(part 1 of 2)
# Autodesk Inventor assembly: PumpConcept.Tube and Pipe Runs
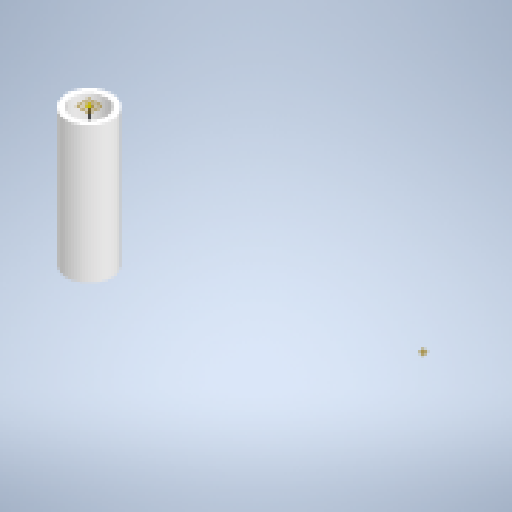
[picture p0: Inventor's stored thumbnail of the model, 512x512]
Saved by Autodesk Inventor 2025.2 (Build 292293000, 293)
## iProperties
Name: ISO 2531 - Flanged Ductile Iron Pipe and Fittings
ActiveState: False
PipeType: Rigid Pipe
RoutePreview: Solid
Material: UnInitValue
Standard: UnInitValue
FittingMaterial: UnInitValue
FittingStandard: UnInitValue
RouteDirection90: True
RouteDirection45: True
DiameterType: Nominal
Diameter: M40
Schedule: PN10
Ending: UnInitValue
IntermediateSegmentsMin: 1000 mm
IntermediateSegmentsMax: 9000 mm
IntermediateSegmentsInc: 10 mm
TerminationSegmentsMin: 1000 mm
TerminationSegmentsMax: 9000 mm
TerminationSegmentsInc: 10 mm
SolidRoutePreviewColor: 12632064
PipingComponentColor: As Material
PipeKey: v3#f52fbdcb-ece8-4303-8b76-5dbe8c7f2f9c#16
Elbow90Key: v3#451ae64e-c79d-4cba-b533-c09b8090ecb2#1
Elbow45Key: v3#81684a3f-f2a4-4fe6-95b1-f067ddead22f#1
_ComponentInfo: <CS><C N="Pipe" R="2.700000" IR="2.000000" PL="PL" PN="ISO 2531 Pipe with Integrally Cast Flanges DN40 PN 10"><CO N="1"><FE V="0"/><FD V="0"/><ET  V="Flanged"/><NS V="M40"/><MA V="0.000000"/><MI V="0.000000"/><WP X="0.000000" Y="-0.000000" Z="0.000000"/><WA X="1.000000" Y="0.000000"  Z="0.000000"/></CO><CO N="2"><FE V="0"/><FD V="1"/><ET V="Flanged"/><NS V="M40"/><MA V="0.000000"/><MI V="0.000000"/><WP X="-50.000000" Y="-0.000000"  Z="0.000000"/><WA X="1.000000" Y="0.000000" Z="0.000000"/></CO></C><C N="Elbow90" ER="14.000000" S1="14.000000" S2="14.000000" D1="0.000000"  D2="0.000000"><CO N="1"><FE V="0"/><FD V="0"/><ET V="Flanged"/><NS V="M40"/><MA V="0.000000"/><MI V="0.000000"/><WP X="14.000000" Y="0.000000"  Z="14.000000"/><WA X="1.000000" Y="0.000000" Z="0.000000"/></CO><CO N="2"><FE V="0"/><FD V="0"/><ET V="Flanged"/><NS V="M40"/><MA V="0.000000"/><MI  V="0.000000"/><WP X="0.000000" Y="0.000000" Z="0.000000"/><WA X="0.000000" Y="0.000000" Z="-1.000000"/></CO></C><C N="Elbow45" ER="33.798990"  S1="14.000000" S2="14.000000" D1="0.000000" D2="0.000000"><CO N="1"><FE V="0"/><FD V="0"/><ET V="Flanged"/><NS V="M40"/><MA V="0.000000"/><MI  V="0.000000"/><WP X="9.899495" Y="0.000000" Z="23.899495"/><WA X="0.707107" Y="0.000000" Z="0.707107"/></CO><CO N="2"><FE V="0"/><FD V="0"/><ET  V="Flanged"/><NS V="M40"/><MA V="0.000000"/><MI V="0.000000"/><WP X="-0.000000" Y="0.000000" Z="-0.000000"/><WA X="-0.000000" Y="0.000000"  Z="-1.000000"/></CO></C></CS>
BendRadius: UnInitValue
CategoryName: UnInitValue
DefaultBendRadius: 80 mm
EndFittingKey: UnInitValue
FlangeKey: UnInitValue
Gap: UnInitValue
GasketKey: UnInitValue
IsButtWelded: UnInitValue
IsFlanged: UnInitValue
MixedUnits: UnInitValue
RoundUpValue: UnInitValue
ShowGap: UnInitValue
StartFittingKey: UnInitValue
SuppressEndFitting: UnInitValue
SuppressStartFitting: UnInitValue
UseFlangsForCouplings: UnInitValue
UseSubASM: UnInitValue
Angle: UnInitValue
CustomFitElbow45Key: UnInitValue
CustomFitElbow90Key: UnInitValue
ElbowCustomKey: UnInitValue
IsSelfDraining: UnInitValue
PipingCustomFitElbowColor: UnInitValue
UseCustomFitElbows: UnInitValue
Name: Hydraulic Hose - Female Taper Thread
PipeType: Flexible Hose
RouteDirection90: UnInitValue
RouteDirection45: UnInitValue
Diameter: 1/2
Schedule: ID=0.5
OD: 2.235200000000000e+000
ID: 1.270000000000000e+000
IntermediateSegmentsMin: UnInitValue
IntermediateSegmentsMax: UnInitValue
IntermediateSegmentsInc: UnInitValue
TerminationSegmentsMin: UnInitValue
TerminationSegmentsMax: UnInitValue
TerminationSegmentsInc: UnInitValue
RoundUpValue: 0.125 in
PipeKey: v3#d489867e-ac9b-47ea-b952-0a1b885f66be#4
CouplingKey: UnInitValue
Elbow90Key: UnInitValue
Elbow45Key: UnInitValue
_ComponentInfo: <CS><C N="Pipe" R="1.117600" OR="1.117600" IR="0.635000" PL="PL" PartType="" SymKey="" PN="Parker Hydraulic Hose - No Skive 1/2"><CO N="1"><FE V="0"/><FD V="0"/><ET V="Hose - Permanent"/><NS V="1/2"/><MA V="2.540000"/><MI V="0.508000"/><WP X="12.700000" Y="0.000000" Z="0.000000"/><WA X="1.000000" Y="0.000000" Z="0.000000"/></CO><CO N="2"><FE V="0"/><FD V="1"/><ET V="Hose - Permanent"/><NS V="1/2"/><MA V="2.540000"/><MI V="0.508000"/><WP X="0.000000" Y="0.000000" Z="0.000000"/><WA X="1.000000" Y="0.000000" Z="0.000000"/></CO></C><C N="StartFitting" PartType="COUPLING" SymKey="COSC"><CO N="1"><FE V="1"/><FD V="1"/><ET V="Threaded"/><NS V="1/2"/><MA V="0.812800"/><MI V="0.162560"/><WP X="0.000000" Y="0.000000" Z="0.000000"/><WA X="1.000000" Y="-0.000000" Z="0.000000"/></CO><CO N="2"><FE V="1"/><FD V="0"/><ET V="Hose - Permanent"/><NS V="1/2"/><MA V="3.200400"/><MI V="3.200400"/><WP X="6.654800" Y="0.000000" Z="0.000000"/><WA X="1.000000" Y="-0.000000" Z="0.000000"/></CO></C><C N="EndFitting" PartType="COUPLING" SymKey="COSC"><CO N="1"><FE V="1"/><FD V="1"/><ET V="Threaded"/><NS V="1/2"/><MA V="0.812800"/><MI V="0.162560"/><WP X="0.000000" Y="0.000000" Z="0.000000"/><WA X="1.000000" Y="-0.000000" Z="0.000000"/></CO><CO N="2"><FE V="1"/><FD V="0"/><ET V="Hose - Permanent"/><NS V="1/2"/><MA V="3.200400"/><MI V="3.200400"/><WP X="6.654800" Y="0.000000" Z="0.000000"/><WA X="1.000000" Y="-0.000000" Z="0.000000"/></CO></C></CS>
BendRadius: 0.500 in
StartFittingKey: v3#cc3bd835-95a2-497d-9893-176cd9c426f6#7
EndFittingKey: v3#cc3bd835-95a2-497d-9893-176cd9c426f6#7
SuppressStartFitting: False
SuppressEndFitting: False
UseSubASM: True
DefaultBendRadius: UnInitValue
Name: JIS G 3458/JIS B 2316 -  Welded Steel Pipe and Fittings
Schedule: 80
IntermediateSegmentsMin: 60 mm
IntermediateSegmentsMax: 5000 mm
IntermediateSegmentsInc: 1 mm
TerminationSegmentsMin: 60 mm
TerminationSegmentsMax: 5000 mm
TerminationSegmentsInc: 1 mm
PipeKey: v3#da14b0ab-0b36-4851-8d66-8c9cd0bcbe86#23
CouplingKey: v3#12b64993-10e6-4915-8315-0c0cce209ad0#8
Elbow90Key: v3#1f65ece3-c41a-48d4-8661-909ed34ade86#8
Elbow45Key: v3#28e76e79-e22c-40ab-8be2-ff545b1407c5#8
_ComponentInfo: <CS><C N="Pipe" R="2.430000" IR="1.920000" PL="PL" PN="JIS G 3458 Pipe 40 A x Sch 80"><CO N="1"><FE V="0"/><FD V="1"/><ET V="Welded"/><NS  V="M40"/><MA V="0.000000"/><MI V="0.000000"/><WP X="0.000000" Y="0.000000" Z="0.000000"/><WA X="-1.000000" Y="0.000000" Z="0.000000"/></CO><CO  N="2"><FE V="0"/><FD V="0"/><ET V="Welded"/><NS V="M40"/><MA V="0.000000"/><MI V="0.000000"/><WP X="-25.000000" Y="0.000000" Z="0.000000"/><WA  X="-1.000000" Y="0.000000" Z="0.000000"/></CO></C><C N="Coupling" CW="3.810000"><CO N="1"><FE V="1"/><FD V="1"/><ET V="Welded"/><NS V="M40"/><MA  V="1.270000"/><MI V="0.254000"/><WP X="-0.000000" Y="0.000000" Z="0.000000"/><WA X="1.000000" Y="0.000000" Z="0.000000"/></CO><CO N="2"><FE  V="1"/><FD V="0"/><ET V="Welded"/><NS V="M40"/><MA V="1.270000"/><MI V="0.254000"/><WP X="3.810000" Y="0.000000" Z="0.000000"/><WA X="1.000000"  Y="0.000000" Z="0.000000"/></CO></C><C N="Elbow90" ER="3.180000" S1="4.450000" S2="4.450000" D1="1.270000" D2="1.270000"><CO N="1"><FE V="1"/><FD  V="1"/><ET V="Welded"/><NS V="M40"/><MA V="1.270000"/><MI V="0.254000"/><WP X="4.450000" Y="-0.000000" Z="4.450000"/><WA X="-1.000000" Y="0.000000"  Z="0.000000"/></CO><CO N="2"><FE V="1"/><FD V="1"/><ET V="Welded"/><NS V="M40"/><MA V="1.270000"/><MI V="0.254000"/><WP X="0.000000" Y="0.000000"  Z="0.000000"/><WA X="0.000000" Y="0.000000" Z="1.000000"/></CO></C><C N="Elbow45" ER="4.973280" S1="3.330000" S2="3.330000" D1="1.270000"  D2="1.270000"><CO N="1"><FE V="1"/><FD V="0"/><ET V="Welded"/><NS V="M40"/><MA V="1.270000"/><MI V="0.254000"/><WP X="2.354666" Y="0.000000"  Z="5.684666"/><WA X="0.707107" Y="0.000000" Z="0.707107"/></CO><CO N="2"><FE V="1"/><FD V="0"/><ET V="Welded"/><NS V="M40"/><MA V="1.270000"/><MI  V="0.254000"/><WP X="0.000000" Y="0.000000" Z="0.000000"/><WA X="0.000000" Y="0.000000" Z="-1.000000"/></CO></C></CS>
USE_R9_BOM: False
Name: Hydraulic Hose - SAE Flanged Connection
_ComponentInfo: <CS><C N="Pipe" R="1.117600" OR="1.117600" IR="0.635000" PL="PL" PartType="" SymKey="" PN="Parker Hydraulic Hose - No Skive 1/2"><CO N="1"><FE V="0"/><FD V="0"/><ET V="Hose - Permanent"/><NS V="1/2"/><MA V="2.540000"/><MI V="0.508000"/><WP X="12.700000" Y="0.000000" Z="0.000000"/><WA X="1.000000" Y="0.000000" Z="0.000000"/></CO><CO N="2"><FE V="0"/><FD V="1"/><ET V="Hose - Permanent"/><NS V="1/2"/><MA V="2.540000"/><MI V="0.508000"/><WP X="0.000000" Y="0.000000" Z="0.000000"/><WA X="1.000000" Y="0.000000" Z="0.000000"/></CO></C><C N="StartFitting" PartType="MISC-HYGENIC" SymKey="ADMF"><CO N="1"><FE V="0"/><FD V="1"/><ET V="Flanged"/><NS V="1/2"/><MA V="0.000000"/><MI V="0.000000"/><WP X="0.000000" Y="0.000000" Z="0.000000"/><WA X="1.000000" Y="0.000000" Z="0.000000"/></CO><CO N="2"><FE V="1"/><FD V="0"/><ET V="Hose - Permanent"/><NS V="1/2"/><MA V="3.200000"/><MI V="3.200000"/><WP X="8.800000" Y="0.000000" Z="0.000000"/><WA X="1.000000" Y="0.000000" Z="0.000000"/></CO></C><C N="EndFitting" PartType="MISC-HYGENIC" SymKey="ADMF"><CO N="1"><FE V="0"/><FD V="1"/><ET V="Flanged"/><NS V="1/2"/><MA V="0.000000"/><MI V="0.000000"/><WP X="0.000000" Y="0.000000" Z="0.000000"/><WA X="1.000000" Y="0.000000" Z="0.000000"/></CO><CO N="2"><FE V="1"/><FD V="0"/><ET V="Hose - Permanent"/><NS V="1/2"/><MA V="3.200000"/><MI V="3.200000"/><WP X="8.800000" Y="0.000000" Z="0.000000"/><WA X="1.000000" Y="0.000000" Z="0.000000"/></CO></C></CS>
StartFittingKey: v3#933069c9-73b6-4141-af99-628d4a97b2c2#1
EndFittingKey: v3#933069c9-73b6-4141-af99-628d4a97b2c2#1
DefaultBendRadius: 12 in
Diameter: 6
Elbow90Key: v3#97ecdcaf-8aa3-4fb0-8b6a-3da783de2ad5#108
Gap: 0.062 in
ID: UnInitValue
IntermediateSegmentsInc: 0.00001 in
IntermediateSegmentsMax: 200 in
IntermediateSegmentsMin: 3 in
IsButtWelded: True
IsFlanged: False
Name: ASTM A 53/A-ASME B16.9 - Steel Butt Welded Pipe
OD: UnInitValue
PipeKey: v3#4ce5e9fa-6da0-4801-ac02-ee7a0fb518d6#77
RouteDirection45: False
Schedule: 40
ShowGap: True
TerminationSegmentsInc: 0.00001 in
TerminationSegmentsMax: 200 in
TerminationSegmentsMin: 3 in
_ComponentInfo: <CS><C N="Elbow90" ER="15.240000" S1="15.240000" S2="15.240000" D1="0.000000" D2="0.000000" PartType="fitting" SymKey="ELBW"><CO N="1"><FE V="2"/><FD V="0"/><ET V="Butt Welded"/><NS V="6"/><MA V="0.000000"/><MI V="0.000000"/><WP X="15.240000" Y="0.000000" Z="15.240000"/><WA X="1.000000" Y="0.000000" Z="-0.000000"/></CO><CO N="2"><FE V="2"/><FD V="1"/><ET V="Butt Welded"/><NS V="6"/><MA V="0.000000"/><MI V="0.000000"/><WP X="0.000000" Y="0.000000" Z="0.000000"/><WA X="0.000000" Y="0.000000" Z="1.000000"/></CO></C><C N="Pipe" R="8.413750" OR="8.413750" IR="7.702550" PL="PL" PartType="pipe" SymKey="" PN="ASTM A 53/A 53M Pipe 6 - Schedule 40"><CO N="1"><FE V="2"/><FD V="0"/><ET V="Welded"/><NS V="6"/><MA V="0.000000"/><MI V="0.000000"/><WP X="25.400000" Y="0.000000" Z="0.000000"/><WA X="1.000000" Y="0.000000" Z="0.000000"/></CO><CO N="2"><FE V="2"/><FD V="1"/><ET V="Welded"/><NS V="6"/><MA V="0.000000"/><MI V="0.000000"/><WP X="0.000000" Y="0.000000" Z="0.000000"/><WA X="1.000000" Y="0.000000" Z="0.000000"/></CO></C></CS>
MixedUnits: False
Name: ASTM A53/A53M-ASME B16.11 - Welded Steel Pipe
Material: Steel
Standard: ASTM A 53/A 53M
FittingMaterial: Steel
FittingStandard: ASME B16.11
OD: Undefined
ID: Undefined
IntermediateSegmentsMin: 1 in
IntermediateSegmentsInc: 0.1 in
TerminationSegmentsMin: 1 in
TerminationSegmentsInc: 0.1 in
PipeKey: v3#4ce5e9fa-6da0-4801-ac02-ee7a0fb518d6#7
CouplingKey: v3#ed415c76-4cec-44a3-ba67-72e47bf70384#4
Elbow90Key: v3#82a08401-12d7-413b-b7f9-9cf3b607be7b#4
Elbow45Key: v3#2e5fd082-3851-4eb0-bde1-6c7078a7d72b#4
_ComponentInfo: <CS><C N="Pipe" R="1.066800" IR="0.789940" PL="PL" PN="ASTM A 53/A 53M Pipe 1/2 - Schedule 40"><CO N="1"><FE V="0"/><FD V="0"/><ET V="Welded"/><NS  V="1/2"/><MA V="0.000000"/><MI V="0.000000"/><WP X="25.400000" Y="0.000000" Z="0.000000"/><WA X="1.000000" Y="0.000000" Z="0.000000"/></CO><CO  N="2"><FE V="0"/><FD V="1"/><ET V="Welded"/><NS V="1/2"/><MA V="0.000000"/><MI V="0.000000"/><WP X="0.000000" Y="0.000000" Z="0.000000"/><WA  X="1.000000" Y="0.000000" Z="0.000000"/></CO></C><C N="Coupling" CW="2.895600"><CO N="1"><FE V="1"/><FD V="1"/><ET V="Welded"/><NS V="1/2"/><MA  V="0.965200"/><MI V="0.193040"/><WP X="-0.000000" Y="0.000000" Z="0.000000"/><WA X="1.000000" Y="0.000000" Z="0.000000"/></CO><CO N="2"><FE  V="1"/><FD V="0"/><ET V="Welded"/><NS V="1/2"/><MA V="0.965200"/><MI V="0.193040"/><WP X="2.895600" Y="0.000000" Z="0.000000"/><WA X="1.000000"  Y="0.000000" Z="0.000000"/></CO></C><C N="Elbow90" ER="1.574800" S1="2.540000" S2="2.540000" D1="0.965200" D2="0.965200"><CO N="1"><FE V="1"/><FD  V="1"/><ET V="Welded"/><NS V="1/2"/><MA V="0.965200"/><MI V="0.193040"/><WP X="2.540000" Y="0.000000" Z="2.540000"/><WA X="-1.000000" Y="0.000000"  Z="-0.000000"/></CO><CO N="2"><FE V="1"/><FD V="0"/><ET V="Welded"/><NS V="1/2"/><MA V="0.965200"/><MI V="0.193040"/><WP X="0.000000" Y="0.000000"  Z="0.000000"/><WA X="0.000000" Y="0.000000" Z="-1.000000"/></CO></C><C N="Elbow45" ER="2.698125" S1="2.082800" S2="2.082800" D1="0.965200"  D2="0.965200"><CO N="1"><FE V="1"/><FD V="0"/><ET V="Welded"/><NS V="1/2"/><MA V="0.965200"/><MI V="0.193040"/><WP X="1.472762" Y="0.000000"  Z="3.555562"/><WA X="0.707107" Y="0.000000" Z="0.707107"/></CO><CO N="2"><FE V="1"/><FD V="0"/><ET V="Welded"/><NS V="1/2"/><MA V="0.965200"/><MI  V="0.193040"/><WP X="0.000000" Y="0.000000" Z="0.000000"/><WA X="0.000000" Y="0.000000" Z="-1.000000"/></CO></C></CS>
DefaultBendRadius: 1 in
Name: ASTM D 1785-ASTM D 2466 - Jointed PVC Pipe and Fittings
ActiveState: True
Material: PVC-Piping
Standard: ASTM D 1785
FittingMaterial: PVC-Piping
FittingStandard: ASTM D 2466
IntermediateSegmentsMax: 100 in
TerminationSegmentsMax: 100 in
PipeKey: v3#4bf12049-4375-491b-8f13-d4ee0c517c57#1
CouplingKey: v3#29993622-4c6a-437e-8b8c-43a0846f8735#1
Elbow90Key: v3#25d2a8db-6517-4627-a5a4-9d27e4d26b9b#1
Elbow45Key: v3#d7b5d569-4a12-4d65-ba55-12203d6ac7ed#1
_ComponentInfo: <CS><C N="Pipe" R="1.066800" IR="0.789940" PL="PL" PN="ASTM D 1785 Pipe 1/2 - Schedule 40"><CO N="1"><FE V="0"/><FD V="0"/><ET V="Jointed"/><NS  V="1/2"/><MA V="2.540000"/><MI V="0.508000"/><WP X="127.000000" Y="0.000000" Z="0.000000"/><WA X="1.000000" Y="0.000000" Z="0.000000"/></CO><CO  N="2"><FE V="0"/><FD V="1"/><ET V="Jointed"/><NS V="1/2"/><MA V="2.540000"/><MI V="0.508000"/><WP X="0.000000" Y="0.000000" Z="0.000000"/><WA  X="1.000000" Y="0.000000" Z="0.000000"/></CO></C><C N="Coupling" CW="3.733165"><CO N="1"><FE V="1"/><FD V="0"/><ET V="Jointed"/><NS V="1/2"/><MA  V="1.747520"/><MI V="0.349504"/><WP X="3.733165" Y="0.000000" Z="0.000000"/><WA X="1.000000" Y="0.000000" Z="0.000000"/></CO><CO N="2"><FE V="1"/><FD  V="1"/><ET V="Jointed"/><NS V="1/2"/><MA V="1.747520"/><MI V="0.349504"/><WP X="0.000000" Y="0.000000" Z="0.000000"/><WA X="1.000000" Y="0.000000"  Z="0.000000"/></CO></C><C N="Elbow90" ER="1.270000" S1="3.017520" S2="3.017520" D1="1.747520" D2="1.747520"><CO N="1"><FE V="1"/><FD V="1"/><ET  V="Jointed"/><NS V="1/2"/><MA V="1.747520"/><MI V="0.349504"/><WP X="3.017520" Y="0.000000" Z="3.017520"/><WA X="-1.000000" Y="0.000000"  Z="-0.000000"/></CO><CO N="2"><FE V="1"/><FD V="1"/><ET V="Jointed"/><NS V="1/2"/><MA V="1.747520"/><MI V="0.349504"/><WP X="0.000000" Y="0.000000"  Z="0.000000"/><WA X="0.000000" Y="0.000000" Z="1.000000"/></CO></C><C N="Elbow45" ER="1.533026" S1="2.382520" S2="2.382520" D1="1.747520"  D2="1.747520"><CO N="1"><FE V="1"/><FD V="1"/><ET V="Jointed"/><NS V="1/2"/><MA V="1.747520"/><MI V="0.349504"/><WP X="1.684696" Y="0.000000"  Z="4.067216"/><WA X="-0.707107" Y="0.000000" Z="-0.707107"/></CO><CO N="2"><FE V="1"/><FD V="1"/><ET V="Jointed"/><NS V="1/2"/><MA V="1.747520"/><MI  V="0.349504"/><WP X="0.000000" Y="0.000000" Z="0.000000"/><WA X="0.000000" Y="0.000000" Z="1.000000"/></CO></C></CS>
Created: 2025-05-29
Part Number: PumpConcept.Tube and Pipe Runs
Document SubType Name: Tube & Pipe
Designer: Simon
Manufacturer: Standard
Standards Organization: Custom
Angle: 92.00 deg
DefaultBendRadius: 2 in
Diameter: 1
Elbow45Key: v3#bf26aa2a-f3dd-474c-8758-922a145c2b02#15
Elbow90Key: v3#3e93288f-9bb7-4e46-9d6b-544f8c20ca1c#3
ElbowCustomKey: v3#1f3bd44a-47ab-42f9-b3e0-74afa0c3f0ca#3
Gap: 0.094 in
IntermediateSegmentsMin: 2 in
IsSelfDraining: True
Name: ASME BPE - Butt Welded
PipeKey: v3#b10c956f-6fc6-429e-8056-0864a8581764#35
Schedule: ID=0.87
TerminationSegmentsMin: 2 in
_ComponentInfo: <CS><C N="Pipe" R="1.270000" OR="1.270000" IR="1.104900" PL="PL" PartType="pipe" SymKey="" PN="ASTM A 269 Tube with Welded ends 1 x 0.87"><CO N="1"><FE V="2"/><FD V="1"/><ET V="Welded"/><NS V="1"/><MA V="0.000000"/><MI V="0.000000"/><WP X="0.000000" Y="0.000000" Z="0.000000"/><WA X="1.000000" Y="0.000000" Z="0.000000"/></CO><CO N="2"><FE V="2"/><FD V="0"/><ET V="Welded"/><NS V="1"/><MA V="0.000000"/><MI V="0.000000"/><WP X="25.400000" Y="0.000000" Z="0.000000"/><WA X="1.000000" Y="0.000000" Z="0.000000"/></CO></C> <C N="Elbow90" ER="7.620000" S1="7.620000" S2="7.620000" D1="0.000000" D2="0.000000" PartType="fitting" SymKey="ELBW Elbow-Butt Weld(90 degree and 45 degree)"><CO N="1"><FE V="2"/><FD V="0"/><ET V="Butt Welded"/><NS V="1"/><MA V="0.000000"/><MI V="0.000000"/><WP X="0.000000" Y="0.000000" Z="0.000000"/><WA X="0.000000" Y="0.000000" Z="-1.000000"/></CO><CO N="2"><FE V="2"/><FD V="1"/><ET V="Butt Welded"/><NS V="1"/><MA V="0.000000"/><MI V="0.000000"/><WP X="0.000000" Y="7.620000" Z="7.620000"/><WA X="0.000000" Y="-1.000000" Z="0.000000"/></CO></C> <C N="Elbow45" ER="5.396250" S1="2.235200" S2="2.235200" D1="0.000000" D2="0.000000" PartType="fitting" SymKey="ELBW"><CO N="1"><FE V="2"/><FD V="0"/><ET V="Butt Welded"/><NS V="1"/><MA V="0.000000"/><MI V="0.000000"/><WP X="1.580525" Y="0.000000" Z="3.815725"/><WA X="0.707107" Y="0.000000" Z="0.707107"/></CO><CO N="2"><FE V="2"/><FD V="1"/><ET V="Butt Welded"/><NS V="1"/><MA V="0.000000"/><MI V="0.000000"/><WP X="0.000000" Y="0.000000" Z="0.000000"/><WA X="0.000000" Y="0.000000" Z="1.000000"/></CO></C> <C N="ElbowCustom" ER="7.746829" S1="7.485916" S2="7.481026" D1="0.004890" D2="0.000000" PartType="fitting" SymKey="ELBW Elbow-Butt Weld(90 degree and 45 degree)"><CO N="1"><FE V="2"/><FD V="1"/><ET V="Butt Welded"/><NS V="1"/><MA V="0.000000"/><MI V="0.000000"/><WP X="0.000000" Y="0.000000" Z="0.000000"/><WA X="0.000000" Y="-0.000000" Z="1.000000"/></CO><CO N="2"><FE V="2"/><FD V="0"/><ET V="Butt Welded"/><NS V="1"/><MA V="0.000000"/><MI V="0.000000"/><WP X="0.000000" Y="7.476469" Z="7.747000"/><WA X="0.000000" Y="0.999391" Z="0.034899"/></CO></C> </CS>
Elbow90Key: v3#6a678020-d9d9-4685-bba9-906b9a167083#10
FlangeKey: v3#c11442d2-c568-438f-a870-8ac9b5b636cb#10
GasketKey: v3#2a41914c-f5fb-4682-9c6a-1870d826d3d0#23
IsButtWelded: False
IsFlanged: True
Name: ASTM A 53/A-ASME B16.5 - Flanged Steel Threaded Pipe
PipeKey: v3#c5bd7d28-cdb3-4507-9f3d-c2787d93fe8a#40
_ComponentInfo: <CS><C N="Elbow90" ER="21.590000" S1="21.590000" S2="21.590000" D1="0.000000" D2="0.000000" PartType="fitting" SymKey="ELFL"><CO N="1"><FE V="2"/><FD V="1"/><ET V="Flanged"/><NS V="6"/><MA V="0.000000"/><MI V="0.000000"/><WP X="21.590000" Y="0.000000" Z="21.590000"/><WA X="-1.000000" Y="0.000000" Z="0.000000"/></CO><CO N="2"><FE V="2"/><FD V="0"/><ET V="Flanged"/><NS V="6"/><MA V="0.000000"/><MI V="0.000000"/><WP X="-0.000000" Y="0.000000" Z="-0.000000"/><WA X="-0.000000" Y="0.000000" Z="-1.000000"/></CO></C><C N="Gasket" CW="0.127000" PartType="fitting" SymKey=""><CO N="1"><FE V="2"/><FD V="1"/><ET V="Flanged"/><NS V="6"/><MA V="0.000000"/><MI V="0.000000"/><WP X="-0.000000" Y="0.127000" Z="0.000000"/><WA X="0.000000" Y="-1.000000" Z="0.000000"/></CO><CO N="2"><FE V="2"/><FD V="0"/><ET V="Flanged"/><NS V="6"/><MA V="0.000000"/><MI V="0.000000"/><WP X="-0.000000" Y="-0.000000" Z="0.000000"/><WA X="0.000000" Y="-1.000000" Z="0.000000"/></CO></C><C N="Pipe" R="8.413750" OR="8.413750" IR="7.702550" PL="PL" PartType="pipe" SymKey="" PN="ASTM A 53/A 53M Pipe with Threaded Ends 6 - Schedule 40"><CO N="1"><FE V="0"/><FD V="1"/><ET V="Threaded"/><NS V="6"/><MA V="3.206953"/><MI V="0.641391"/><WP X="7.683500" Y="0.000000" Z="0.000000"/><WA X="-1.000000" Y="0.000000" Z="-0.000000"/></CO><CO N="2"><FE V="0"/><FD V="0"/><ET V="Threaded"/><NS V="6"/><MA V="3.206953"/><MI V="0.641391"/><WP X="0.000000" Y="0.000000" Z="-0.000000"/><WA X="-1.000000" Y="0.000000" Z="-0.000000"/></CO></C><C N="Flange" CW="5.232400" PartType="fitting" SymKey="FLSC"><CO N="1"><FE V="2"/><FD V="1"/><ET V="Flanged"/><NS V="6"/><MA V="0.000000"/><MI V="0.000000"/><WP X="0.000000" Y="0.000000" Z="0.000000"/><WA X="1.000000" Y="0.000000" Z="0.000000"/></CO><CO N="2"><FE V="1"/><FD V="0"/><ET V="Threaded"/><NS V="6"/><MA V="5.232400"/><MI V="1.046480"/><WP X="5.232400" Y="0.000000" Z="0.000000"/><WA X="1.000000" Y="0.000000" Z="0.000000"/></CO></C> </CS>
IsSelfDraining: False
Name: ASME B36.10M-ASME B16.11 - Steel Threaded Pipe
Material: Wrought Steel
Standard: ASME B36.10M
Schedule: 30
OD: 2.1336
ID: 1.651
PipeKey: v3#4a736116-503a-44ad-a922-868ac6b46736#1
CouplingKey: v3#52ad3977-2b89-4007-a6a6-7626bac0ae85#4
Elbow90Key: v3#160eac10-3e6f-4b5c-839c-61eee0d373dc#4
Elbow45Key: v3#5c2ab816-abcb-49a6-a106-4733af000f51#4
_ComponentInfo: <CS><C N="Pipe" R="1.066800" IR="0.825500" PL="PL" PN="ASME B36.10M Pipe with Threaded Ends 1/2 - Schedule 30"><CO N="1"><FE V="0"/><FD V="1"/><ET  V="Threaded"/><NS V="1/2"/><MA V="1.355598"/><MI V="0.271120"/><WP X="25.400000" Y="0.000000" Z="-0.000000"/><WA X="-1.000000" Y="0.000000"  Z="0.000000"/></CO><CO N="2"><FE V="0"/><FD V="0"/><ET V="Threaded"/><NS V="1/2"/><MA V="1.355598"/><MI V="0.271120"/><WP X="0.000000" Y="0.000000"  Z="-0.000000"/><WA X="-1.000000" Y="0.000000" Z="0.000000"/></CO></C><C N="Coupling" CW="4.775200"><CO N="1"><FE V="1"/><FD V="0"/><ET  V="Threaded"/><NS V="1/2"/><MA V="1.355598"/><MI V="0.271120"/><WP X="4.775200" Y="0.000000" Z="0.000000"/><WA X="1.000000" Y="0.000000"  Z="0.000000"/></CO><CO N="2"><FE V="1"/><FD V="1"/><ET V="Threaded"/><NS V="1/2"/><MA V="1.355598"/><MI V="0.271120"/><WP X="0.000000" Y="0.000000"  Z="0.000000"/><WA X="1.000000" Y="0.000000" Z="0.000000"/></CO></C><C N="Elbow90" ER="1.971802" S1="3.327400" S2="3.327400" D1="1.355598"  D2="1.355598"><CO N="1"><FE V="1"/><FD V="1"/><ET V="Threaded"/><NS V="1/2"/><MA V="1.355598"/><MI V="0.271120"/><WP X="3.327400" Y="0.000000"  Z="3.327400"/><WA X="-1.000000" Y="0.000000" Z="0.000000"/></CO><CO N="2"><FE V="1"/><FD V="0"/><ET V="Threaded"/><NS V="1/2"/><MA V="1.355598"/><MI  V="0.271120"/><WP X="-0.000000" Y="0.000000" Z="0.000000"/><WA X="-0.000000" Y="0.000000" Z="-1.000000"/></CO></C><C N="Elbow45" ER="2.859399"  S1="2.540000" S2="2.540000" D1="1.355598" D2="1.355598"><CO N="1"><FE V="1"/><FD V="0"/><ET V="Threaded"/><NS V="1/2"/><MA V="1.355598"/><MI  V="0.271120"/><WP X="1.796051" Y="0.000000" Z="4.336051"/><WA X="0.707107" Y="0.000000" Z="0.707107"/></CO><CO N="2"><FE V="1"/><FD V="1"/><ET  V="Threaded"/><NS V="1/2"/><MA V="1.355598"/><MI V="0.271120"/><WP X="0.000000" Y="0.000000" Z="0.000000"/><WA X="0.000000" Y="0.000000"  Z="1.000000"/></CO></C></CS>
Name: DIN 2458/DIN 2605 - Welded Steel Pipe and Fittings
Schedule: ID=30.7
PipeKey: v3#dcef2839-8903-4c98-a96c-b861f5d9bb7f#98
Elbow90Key: v3#ace818b0-7b7c-4ad9-b19c-6da358a202c1#17
Elbow45Key: v3#97879d80-057e-491b-840b-74a9b3a7cf63#17
_ComponentInfo: <CS><C N="Pipe" R="2.415000" IR="1.535000" PL="PL" PN="DIN 2458 Pipe 48.3 x 8.8"><CO N="1"><FE V="2"/><FD V="0"/><ET V="Welded"/><NS V="M40"/><MA  V="0.000000"/><MI V="0.000000"/><WP X="25.000000" Y="0.000000" Z="0.000000"/><WA X="1.000000" Y="0.000000" Z="0.000000"/></CO><CO N="2"><FE  V="2"/><FD V="1"/><ET V="Welded"/><NS V="M40"/><MA V="0.000000"/><MI V="0.000000"/><WP X="0.000000" Y="0.000000" Z="0.000000"/><WA X="1.000000"  Y="0.000000" Z="0.000000"/></CO></C><C N="Elbow90" ER="3.800000" S1="3.800000" S2="3.800000" D1="0.000000" D2="0.000000"><CO N="1"><FE V="2"/><FD  V="1"/><ET V="Butt Welded"/><NS V="M40"/><MA V="0.000000"/><MI V="0.000000"/><WP X="0.000000" Y="0.000000" Z="0.000000"/><WA X="0.000000" Y="0.000000"  Z="1.000000"/></CO><CO N="2"><FE V="2"/><FD V="0"/><ET V="Butt Welded"/><NS V="M40"/><MA V="0.000000"/><MI V="0.000000"/><WP X="3.800000" Y="0.000000"  Z="3.800000"/><WA X="1.000000" Y="0.000000" Z="-0.000000"/></CO></C><C N="Elbow45" ER="3.862742" S1="1.600000" S2="1.600000" D1="0.000000"  D2="0.000000"><CO N="1"><FE V="2"/><FD V="1"/><ET V="Butt Welded"/><NS V="M40"/><MA V="0.000000"/><MI V="0.000000"/><WP X="0.000000" Y="0.000000"  Z="0.000000"/><WA X="0.000000" Y="0.000000" Z="1.000000"/></CO><CO N="2"><FE V="2"/><FD V="0"/><ET V="Butt Welded"/><NS V="M40"/><MA V="0.000000"/><MI  V="0.000000"/><WP X="1.131371" Y="0.000000" Z="2.731371"/><WA X="0.707107" Y="0.000000" Z="0.707107"/></CO></C></CS>
Name: Hydraulic Hose - Male Taper Thread
_ComponentInfo: <CS><C N="Pipe" R="1.117600" OR="1.117600" IR="0.635000" PL="PL" PartType="" SymKey="" PN="Parker Hydraulic Hose - No Skive 1/2"><CO N="1"><FE V="0"/><FD V="0"/><ET V="Hose - Permanent"/><NS V="1/2"/><MA V="2.540000"/><MI V="0.508000"/><WP X="12.700000" Y="0.000000" Z="0.000000"/><WA X="1.000000" Y="0.000000" Z="0.000000"/></CO><CO N="2"><FE V="0"/><FD V="1"/><ET V="Hose - Permanent"/><NS V="1/2"/><MA V="2.540000"/><MI V="0.508000"/><WP X="0.000000" Y="0.000000" Z="0.000000"/><WA X="1.000000" Y="0.000000" Z="0.000000"/></CO></C><C N="StartFitting" PartType="MISC-HYGENIC" SymKey="ADMF"><CO N="1"><FE V="0"/><FD V="1"/><ET V="Threaded"/><NS V="1/2"/><MA V="1.985010"/><MI V="0.397002"/><WP X="0.000000" Y="0.000000" Z="0.000000"/><WA X="1.000000" Y="0.000000" Z="0.000000"/></CO><CO N="2"><FE V="1"/><FD V="0"/><ET V="Hose - Permanent"/><NS V="1/2"/><MA V="3.200400"/><MI V="3.200400"/><WP X="7.213600" Y="0.000000" Z="0.000000"/><WA X="1.000000" Y="0.000000" Z="0.000000"/></CO></C><C N="EndFitting" PartType="MISC-HYGENIC" SymKey="ADMF"><CO N="1"><FE V="0"/><FD V="1"/><ET V="Threaded"/><NS V="1/2"/><MA V="1.985010"/><MI V="0.397002"/><WP X="0.000000" Y="0.000000" Z="0.000000"/><WA X="1.000000" Y="0.000000" Z="0.000000"/></CO><CO N="2"><FE V="1"/><FD V="0"/><ET V="Hose - Permanent"/><NS V="1/2"/><MA V="3.200400"/><MI V="3.200400"/><WP X="7.213600" Y="0.000000" Z="0.000000"/><WA X="1.000000" Y="0.000000" Z="0.000000"/></CO></C></CS>
StartFittingKey: v3#c8250148-a7b6-458b-b7bd-3b56763ca7cc#13
EndFittingKey: v3#c8250148-a7b6-458b-b7bd-3b56763ca7cc#13
Name: JIS G 3442/JIS B 2301 Threaded Steel Pipe and Iron Fittings
Schedule: ID=16.1
IntermediateSegmentsMin: 20 mm
TerminationSegmentsMin: 20 mm
PipeKey: v3#9964fba4-9d5a-4d75-85a8-e38022ccdce1#2
CouplingKey: v3#181262db-c004-4877-bc40-c64b931a44f6#3
Elbow90Key: v3#6c92b367-65e9-486b-b952-db434ae2548d#3
Elbow45Key: v3#960407aa-00b9-4d72-aae7-d50595845cfd#3
_ComponentInfo: <CS><C N="Pipe" R="1.085000" IR="0.805000" PL="PL" PN="JIS G 3442 Pipe with Threaded Ends 21.7 x 2.8"><CO N="1"><FE V="0"/><FD V="1"/><ET V="Threaded"/><NS V="1/2"/><MA V="1.316000"/><MI V="0.263200"/><WP X="25.000000" Y="0.000000" Z="-0.000000"/><WA X="-1.000000" Y="0.000000" Z="0.000000"/></CO><CO N="2"><FE V="0"/><FD V="0"/><ET V="Threaded"/><NS V="1/2"/><MA V="1.316000"/><MI V="0.263200"/><WP X="0.000000" Y="0.000000" Z="0.000000"/><WA X="-1.000000" Y="0.000000" Z="0.000000"/></CO></C><C N="Coupling" CW="3.500000"><CO N="1"><FE V="1"/><FD V="1"/><ET V="Threaded"/><NS V="1/2"/><MA V="1.100000"/><MI V="0.220000"/><WP X="0.000000" Y="-0.000000" Z="0.000000"/><WA X="1.000000" Y="0.000000" Z="0.000000"/></CO><CO N="2"><FE V="1"/><FD V="0"/><ET V="Threaded"/><NS V="1/2"/><MA V="1.100000"/><MI V="0.220000"/><WP X="3.500000" Y="0.000000" Z="0.000000"/><WA X="1.000000" Y="0.000000" Z="0.000000"/></CO></C><C N="Elbow90" ER="1.600000" S1="2.700000" S2="2.700000" D1="1.100000" D2="1.100000"><CO N="1"><FE V="1"/><FD V="0"/><ET V="Threaded"/><NS V="1/2"/><MA V="1.100000"/><MI V="0.220000"/><WP X="-0.000000" Y="0.000000" Z="-0.000000"/><WA X="-0.000000" Y="0.000000" Z="-1.000000"/></CO><CO N="2"><FE V="1"/><FD V="1"/><ET V="Threaded"/><NS V="1/2"/><MA V="1.100000"/><MI V="0.220000"/><WP X="2.700000" Y="0.000000" Z="2.700000"/><WA X="-1.000000" Y="0.000000" Z="0.000000"/></CO></C><C N="Elbow45" ER="2.414214" S1="2.100000" S2="2.100000" D1="1.100000" D2="1.100000"><CO N="1"><FE V="1"/><FD V="0"/><ET V="Threaded"/><NS V="1/2"/><MA V="1.100000"/><MI V="0.220000"/><WP X="0.000000" Y="0.000000" Z="0.000000"/><WA X="0.000000" Y="0.000000" Z="-1.000000"/></CO><CO N="2"><FE V="1"/><FD V="1"/><ET V="Threaded"/><NS V="1/2"/><MA V="1.100000"/><MI V="0.220000"/><WP X="1.484924" Y="0.000000" Z="3.584924"/><WA X="-0.707107" Y="0.000000" Z="-0.707107"/></CO></C></CS>
DefaultBendRadius: 25.4 mm
Name: ASTM B 88-ASME B16.22 - Soldered Copper Tubing
PipeType: Tubing
Material: Copper
Standard: ASTM B 88
FittingMaterial: *
FittingStandard: ASME B16.22
Schedule: L
IntermediateSegmentsMin: 0.000 in
IntermediateSegmentsMax: 100.000 in
IntermediateSegmentsInc: 0.100 in
TerminationSegmentsMin: 0.000 in
TerminationSegmentsMax: 100.000 in
TerminationSegmentsInc: 0.100 in
SolidRoutePreviewColor: 49344
PipeKey: v3#44b182c9-4bce-4825-bb4d-596143122252#7
CouplingKey: v3#0dc1ae02-7bbf-4ccf-8498-581434b0a765#3
_ComponentInfo: <CS><C N="Pipe" R="0.793750" IR="0.692150" PL="PL" PN="ASTM B 88 Tube 1/2 - Type L"><CO N="1"><FE V="0"/><FD V="0"/><ET V="Soldered"/><NS V="1/2"/><MA V="2.540000"/><MI V="0.508000"/><WP X="254.000000" Y="0.000000" Z="0.000000"/><WA X="1.000000" Y="0.000000" Z="0.000000"/></CO><CO N="2"><FE V="0"/><FD V="1"/><ET V="Soldered"/><NS V="1/2"/><MA V="2.540000"/><MI V="0.508000"/><WP X="0.000000" Y="0.000000" Z="0.000000"/><WA X="1.000000" Y="0.000000" Z="0.000000"/></CO></C><C N="Coupling" CW="2.540000"><CO N="1"><FE V="1"/><FD V="1"/><ET V="Soldered"/><NS V="1/2"/><MA V="1.270000"/><MI V="0.254000"/><WP X="2.540000" Y="0.000000" Z="-0.000000"/><WA X="-1.000000" Y="0.000000" Z="0.000000"/></CO><CO N="2"><FE V="1"/><FD V="0"/><ET V="Soldered"/><NS V="1/2"/><MA V="1.270000"/><MI V="0.254000"/><WP X="0.000000" Y="0.000000" Z="0.000000"/><WA X="-1.000000" Y="0.000000" Z="0.000000"/></CO></C></CS>
DefaultBendRadius: 2.000 in
CustomFitElbow90Key: v3#0eccf1d3-7418-433e-bb0f-cd3ee6f3b39a#119
Elbow90Key: v3#97ecdcaf-8aa3-4fb0-8b6a-3da783de2ad5#119
Name: ASTM A 53/A-ASME B16.9 - Steel Butt Welded Pipe (Custom Elbows)
UseCustomFitElbows: True
_ComponentInfo: <CS><C N="Pipe" R="8.413750" OR="8.413750" IR="7.702550" PL="PL" PartType="pipe" SymKey="" PN="ASTM A 53/A 53M Pipe 6 - Schedule 40"><CO N="1"><FE V="2"/><FD V="0"/><ET V="Welded"/><NS V="6"/><MA V="0.000000"/><MI V="0.000000"/><WP X="25.400000" Y="0.000000" Z="0.000000"/><WA X="1.000000" Y="0.000000" Z="0.000000"/></CO><CO N="2"><FE V="2"/><FD V="1"/><ET V="Welded"/><NS V="6"/><MA V="0.000000"/><MI V="0.000000"/><WP X="0.000000" Y="0.000000" Z="0.000000"/><WA X="1.000000" Y="0.000000" Z="0.000000"/></CO></C><C N="Elbow90" ER="15.240000" S1="15.240000" S2="15.240000" D1="0.000000" D2="0.000000" PartType="fitting" SymKey="ELBW"><CO N="1"><FE V="2"/><FD V="0"/><ET V="Butt Welded"/><NS V="6"/><MA V="0.000000"/><MI V="0.000000"/><WP X="15.240000" Y="0.000000" Z="15.240000"/><WA X="1.000000" Y="0.000000" Z="-0.000000"/></CO><CO N="2"><FE V="2"/><FD V="1"/><ET V="Butt Welded"/><NS V="6"/><MA V="0.000000"/><MI V="0.000000"/><WP X="0.000000" Y="0.000000" Z="0.000000"/><WA X="0.000000" Y="0.000000" Z="1.000000"/></CO></C> <C N="CustomFitElbow90" ER="15.240000" S1="15.240000" S2="15.240000" D1="0.000000" D2="0.000000" PartType="fitting" SymKey="ELBW"><CO N="1"><FE V="2"/><FD V="0"/><ET V="Butt Welded"/><NS V="6"/><MA V="0.000000"/><MI V="0.000000"/><WP X="15.240000" Y="0.000000" Z="15.240000"/><WA X="1.000000" Y="0.000000" Z="-0.000000"/></CO><CO N="2"><FE V="2"/><FD V="1"/><ET V="Butt Welded"/><NS V="6"/><MA V="0.000000"/><MI V="0.000000"/><WP X="0.000000" Y="0.000000" Z="0.000000"/><WA X="0.000000" Y="0.000000" Z="1.000000"/></CO></C> </CS>
PipingCustomFitElbowColor: As Material
FlangeKey: v3#24991861-26e3-4c21-a713-f46e314eddd5#10
Name: ASTM A 53/A 53M - Butt Welded/Flanged Steel Pipe
UseFlangsForCouplings: False
_ComponentInfo: <CS><C N="Pipe" R="8.413750" OR="8.413750" IR="7.702550" PL="PL" PartType="pipe" SymKey="" PN="ASTM A 53/A 53M Pipe 6 - Schedule 40"><CO N="1"><FE V="2"/><FD V="0"/><ET V="Welded"/><NS V="6"/><MA V="0.000000"/><MI V="0.000000"/><WP X="25.400000" Y="0.000000" Z="0.000000"/><WA X="1.000000" Y="0.000000" Z="0.000000"/></CO><CO N="2"><FE V="2"/><FD V="1"/><ET V="Welded"/><NS V="6"/><MA V="0.000000"/><MI V="0.000000"/><WP X="0.000000" Y="0.000000" Z="0.000000"/><WA X="1.000000" Y="0.000000" Z="0.000000"/></CO></C> <C N="Elbow90" ER="21.590000" S1="21.590000" S2="21.590000" D1="0.000000" D2="0.000000" PartType="fitting" SymKey="ELFL"><CO N="1"><FE V="2"/><FD V="1"/><ET V="Flanged"/><NS V="6"/><MA V="0.000000"/><MI V="0.000000"/><WP X="21.590000" Y="0.000000" Z="21.590000"/><WA X="-1.000000" Y="0.000000" Z="0.000000"/></CO><CO N="2"><FE V="2"/><FD V="0"/><ET V="Flanged"/><NS V="6"/><MA V="0.000000"/><MI V="0.000000"/><WP X="-0.000000" Y="0.000000" Z="-0.000000"/><WA X="-0.000000" Y="0.000000" Z="-1.000000"/></CO></C> <C N="Gasket" CW="0.127000" PartType="fitting" SymKey=""><CO N="1"><FE V="2"/><FD V="1"/><ET V="Flanged"/><NS V="6"/><MA V="0.000000"/><MI V="0.000000"/><WP X="-0.000000" Y="0.127000" Z="0.000000"/><WA X="0.000000" Y="-1.000000" Z="0.000000"/></CO><CO N="2"><FE V="2"/><FD V="0"/><ET V="Flanged"/><NS V="6"/><MA V="0.000000"/><MI V="0.000000"/><WP X="-0.000000" Y="-0.000000" Z="0.000000"/><WA X="0.000000" Y="-1.000000" Z="0.000000"/></CO></C> <C N="Flange" CW="9.855200" PartType="fitting" SymKey="FLWN"><CO N="1"><FE V="2"/><FD V="1"/><ET V="Flanged"/><NS V="6"/><MA V="0.000000"/><MI V="0.000000"/><WP X="0.000000" Y="-0.000000" Z="0.000000"/><WA X="1.000000" Y="0.000000" Z="0.000000"/></CO><CO N="2"><FE V="2"/><FD V="0"/><ET V="Butt Welded"/><NS V="6"/><MA V="0.000000"/><MI V="0.000000"/><WP X="9.855200" Y="0.000000" Z="0.000000"/><WA X="1.000000" Y="0.000000" Z="0.000000"/></CO></C> </CS>
Name: ISO 7598/ISO 49 - Threaded Steel Pipe with Iron Fittings
IntermediateSegmentsMin: 50.8 mm
IntermediateSegmentsMax: 5080 mm
IntermediateSegmentsInc: 2.54 mm
TerminationSegmentsMin: 50.8 mm
TerminationSegmentsMax: 5080 mm
TerminationSegmentsInc: 2.54 mm
PipeKey: v3#1052637f-74b5-47f4-adeb-d4e8d3fa53b8#1
CouplingKey: v3#7e56b2cb-a132-4546-b8a7-a14538454b94#3
Elbow90Key: v3#b72bb08b-ad33-47cc-a03d-7f3d76c6616b#3
Elbow45Key: v3#a96c5204-26e4-4bb2-b8f1-f0623fbc94bb#2
_ComponentInfo: <CS><C N="Pipe" R="1.065000" IR="0.805000" PL="PL" PN="ISO 7598 Tube with Threaded Ends DN15"><CO N="1"><FE V="0"/><FD V="1"/><ET V="Threaded"/><NS V="1/2"/><MA V="1.316000"/><MI V="0.263200"/><WP X="25.000000" Y="0.000000" Z="-0.000000"/><WA X="-1.000000" Y="0.000000" Z="0.000000"/></CO><CO N="2"><FE V="0"/><FD V="0"/><ET V="Threaded"/><NS V="1/2"/><MA V="1.316000"/><MI V="0.263200"/><WP X="0.000000" Y="0.000000" Z="0.000000"/><WA X="-1.000000" Y="0.000000" Z="0.000000"/></CO></C><C N="Coupling" CW="3.600000"><CO N="1"><FE V="1"/><FD V="0"/><ET V="Threaded"/><NS V="1/2"/><MA V="1.300000"/><MI V="0.260000"/><WP X="3.600000" Y="0.000000" Z="0.000000"/><WA X="1.000000" Y="0.000000" Z="0.000000"/></CO><CO N="2"><FE V="1"/><FD V="1"/><ET V="Threaded"/><NS V="1/2"/><MA V="1.300000"/><MI V="0.260000"/><WP X="-0.000000" Y="0.000000" Z="0.000000"/><WA X="1.000000" Y="-0.000000" Z="0.000000"/></CO></C><C N="Elbow90" ER="4.200000" S1="5.500000" S2="5.500000" D1="1.300000" D2="1.300000"><CO N="1"><FE V="1"/><FD V="1"/><ET V="Threaded"/><NS V="1/2"/><MA V="1.300000"/><MI V="0.260000"/><WP X="5.500000" Y="0.000000" Z="5.500000"/><WA X="-1.000000" Y="0.000000" Z="0.000000"/></CO><CO N="2"><FE V="1"/><FD V="0"/><ET V="Threaded"/><NS V="1/2"/><MA V="1.300000"/><MI V="0.260000"/><WP X="-0.000000" Y="0.000000" Z="-0.000000"/><WA X="-0.000000" Y="0.000000" Z="-1.000000"/></CO></C><C N="Elbow45" ER="5.552691" S1="3.600000" S2="3.600000" D1="1.300000" D2="1.300000"><CO N="1"><FE V="1"/><FD V="1"/><ET V="Threaded"/><NS V="1/2"/><MA V="1.300000"/><MI V="0.260000"/><WP X="2.545584" Y="0.000000" Z="6.145584"/><WA X="-0.707107" Y="0.000000" Z="-0.707107"/></CO><CO N="2"><FE V="1"/><FD V="0"/><ET V="Threaded"/><NS V="1/2"/><MA V="1.300000"/><MI V="0.260000"/><WP X="-0.000000" Y="0.000000" Z="-0.000000"/><WA X="-0.000000" Y="0.000000" Z="-1.000000"/></CO></C></CS>
Name: ANSI/ASME B36.19M-ASME B16.3 - Threaded Pipe with Iron Fittings
Material: Stainless Steel
Standard: ANSI/ASME B36.19M
FittingMaterial: Malleable Iron
FittingStandard: ASME B16.3
Schedule: 40S
PipeKey: v3#323c0148-c750-449d-a0c6-11721f2a5046#1
CouplingKey: v3#771d4942-b9e7-43bc-9d41-ab12a9580492#3
Elbow90Key: v3#bc6b44ab-9235-4590-b699-74498030a1ff#3
Elbow45Key: v3#626cc28c-1a24-4045-be0d-40d896dc828d#3
_ComponentInfo: <CS><C N="Pipe" R="1.066800" IR="0.789940" PL="PL" PN="ANSI/ASME B36.19M Pipe with Threaded Ends 1/2 - Schedule 40S"><CO N="1"><FE V="0"/><FD  V="1"/><ET V="Threaded"/><NS V="1/2"/><MA V="1.355598"/><MI V="0.271120"/><WP X="25.400000" Y="0.000000" Z="-0.000000"/><WA X="-1.000000"  Y="0.000000" Z="0.000000"/></CO><CO N="2"><FE V="0"/><FD V="0"/><ET V="Threaded"/><NS V="1/2"/><MA V="1.355598"/><MI V="0.271120"/><WP X="0.000000"  Y="0.000000" Z="-0.000000"/><WA X="-1.000000" Y="0.000000" Z="0.000000"/></CO></C><C N="Coupling" CW="3.403600"><CO N="1"><FE V="1"/><FD V="0"/><ET  V="Threaded"/><NS V="1/2"/><MA V="1.092200"/><MI V="0.218440"/><WP X="3.403600" Y="-0.000000" Z="0.000000"/><WA X="1.000000" Y="-0.000000"  Z="0.000000"/></CO><CO N="2"><FE V="1"/><FD V="1"/><ET V="Threaded"/><NS V="1/2"/><MA V="1.092200"/><MI V="0.218440"/><WP X="0.000000" Y="-0.000000"  Z="0.000000"/><WA X="1.000000" Y="-0.000000" Z="0.000000"/></CO></C><C N="Elbow90" ER="1.752600" S1="2.844800" S2="2.844800" D1="1.092200"  D2="1.092200"><CO N="1"><FE V="1"/><FD V="1"/><ET V="Threaded"/><NS V="1/2"/><MA V="1.092200"/><MI V="0.218440"/><WP X="2.844800" Y="0.000000"  Z="2.844800"/><WA X="-1.000000" Y="0.000000" Z="0.000000"/></CO><CO N="2"><FE V="1"/><FD V="0"/><ET V="Threaded"/><NS V="1/2"/><MA V="1.092200"/><MI  V="0.218440"/><WP X="0.000000" Y="0.000000" Z="-0.000000"/><WA X="-0.000000" Y="0.000000" Z="-1.000000"/></CO></C><C N="Elbow45" ER="2.759446"  S1="2.235200" S2="2.235200" D1="1.092200" D2="1.092200"><CO N="1"><FE V="1"/><FD V="1"/><ET V="Threaded"/><NS V="1/2"/><MA V="1.092200"/><MI  V="0.218440"/><WP X="1.580525" Y="0.000000" Z="3.815725"/><WA X="-0.707107" Y="0.000000" Z="-0.707107"/></CO><CO N="2"><FE V="1"/><FD V="0"/><ET  V="Threaded"/><NS V="1/2"/><MA V="1.092200"/><MI V="0.218440"/><WP X="0.000000" Y="0.000000" Z="-0.000000"/><WA X="-0.000000" Y="0.000000"  Z="-1.000000"/></CO></C></CS>
Name: DIN 2458/DIN EN 10242 - Threaded Steel Pipe and Iron Fittings
Schedule: ID=12.3
PipeKey: v3#d689fd5f-ac5a-46d7-a883-3089b2f6e0a4#28
CouplingKey: v3#d2599e7a-1865-48da-a234-5418a1cd5dfe#3
Elbow90Key: v3#9fba244e-81ed-4fc6-a9ac-7eb372fa3ffe#3
Elbow45Key: v3#6ce5b1be-37aa-4928-b23a-0df64e6ddf38#2
_ComponentInfo: <CS><C N="Pipe" R="1.065000" IR="0.615000" PL="PL" PN="DIN 2458 Pipe with Threaded Ends 21.3 x 4.5"><CO N="1"><FE V="0"/><FD V="1"/><ET V="Threaded"/><NS V="1/2"/><MA V="1.372000"/><MI V="0.274400"/><WP X="25.000000" Y="0.000000" Z="-0.000000"/><WA X="-1.000000" Y="0.000000" Z="0.000000"/></CO><CO N="2"><FE V="0"/><FD V="0"/><ET V="Threaded"/><NS V="1/2"/><MA V="1.372000"/><MI V="0.274400"/><WP X="-0.000000" Y="0.000000" Z="-0.000000"/><WA X="-1.000000" Y="0.000000" Z="0.000000"/></CO></C><C N="Coupling" CW="3.600000"><CO N="1"><FE V="1"/><FD V="1"/><ET V="Threaded"/><NS V="1/2"/><MA V="1.300000"/><MI V="0.260000"/><WP X="0.000000" Y="0.000000" Z="0.000000"/><WA X="1.000000" Y="0.000000" Z="0.000000"/></CO><CO N="2"><FE V="1"/><FD V="0"/><ET V="Threaded"/><NS V="1/2"/><MA V="1.300000"/><MI V="0.260000"/><WP X="3.600000" Y="0.000000" Z="0.000000"/><WA X="1.000000" Y="0.000000" Z="0.000000"/></CO></C><C N="Elbow90" ER="4.200000" S1="5.500000" S2="5.500000" D1="1.300000" D2="1.300000"><CO N="1"><FE V="1"/><FD V="0"/><ET V="Threaded"/><NS V="1/2"/><MA V="1.300000"/><MI V="0.260000"/><WP X="-0.000000" Y="0.000000" Z="-0.000000"/><WA X="-0.000000" Y="0.000000" Z="-1.000000"/></CO><CO N="2"><FE V="1"/><FD V="1"/><ET V="Threaded"/><NS V="1/2"/><MA V="1.300000"/><MI V="0.260000"/><WP X="5.500000" Y="0.000000" Z="5.500000"/><WA X="-1.000000" Y="0.000000" Z="0.000000"/></CO></C><C N="Elbow45" ER="5.552691" S1="3.600000" S2="3.600000" D1="1.300000" D2="1.300000"><CO N="1"><FE V="1"/><FD V="1"/><ET V="Threaded"/><NS V="1/2"/><MA V="1.300000"/><MI V="0.260000"/><WP X="2.545584" Y="0.000000" Z="6.145584"/><WA X="-0.707107" Y="0.000000" Z="-0.707107"/></CO><CO N="2"><FE V="1"/><FD V="0"/><ET V="Threaded"/><NS V="1/2"/><MA V="1.300000"/><MI V="0.260000"/><WP X="-0.000000" Y="0.000000" Z="-0.000000"/><WA X="-0.000000" Y="0.000000" Z="-1.000000"/></CO></C></CS>
Name: Hydraulic Hose - Female Thread - Swivel
_ComponentInfo: <CS><C N="Pipe" R="1.117600" OR="1.117600" IR="0.635000" PL="PL" PartType="" SymKey="" PN="Parker Hydraulic Hose - No Skive 1/2"><CO N="1"><FE V="0"/><FD V="0"/><ET V="Hose - Permanent"/><NS V="1/2"/><MA V="2.540000"/><MI V="0.508000"/><WP X="12.700000" Y="0.000000" Z="0.000000"/><WA X="1.000000" Y="0.000000" Z="0.000000"/></CO><CO N="2"><FE V="0"/><FD V="1"/><ET V="Hose - Permanent"/><NS V="1/2"/><MA V="2.540000"/><MI V="0.508000"/><WP X="0.000000" Y="0.000000" Z="0.000000"/><WA X="1.000000" Y="0.000000" Z="0.000000"/></CO></C><C N="StartFitting" PartType="COUPLING" SymKey="COSC"><CO N="1"><FE V="1"/><FD V="1"/><ET V="Threaded"/><NS V="3/4-16 UNF"/><MA V="0.970000"/><MI V="0.194000"/><WP X="-0.000000" Y="0.000000" Z="0.000000"/><WA X="1.000000" Y="0.000000" Z="0.000000"/></CO><CO N="2"><FE V="1"/><FD V="0"/><ET V="Hose - Permanent"/><NS V="1/2"/><MA V="3.470000"/><MI V="3.470000"/><WP X="6.650000" Y="0.000000" Z="0.000000"/><WA X="1.000000" Y="0.000000" Z="0.000000"/></CO></C><C N="EndFitting" PartType="COUPLING" SymKey="COSC"><CO N="1"><FE V="1"/><FD V="1"/><ET V="Threaded"/><NS V="3/4-16 UNF"/><MA V="0.970000"/><MI V="0.194000"/><WP X="-0.000000" Y="0.000000" Z="0.000000"/><WA X="1.000000" Y="0.000000" Z="0.000000"/></CO><CO N="2"><FE V="1"/><FD V="0"/><ET V="Hose - Permanent"/><NS V="1/2"/><MA V="3.470000"/><MI V="3.470000"/><WP X="6.650000" Y="0.000000" Z="0.000000"/><WA X="1.000000" Y="0.000000" Z="0.000000"/></CO></C></CS>
StartFittingKey: v3#c5e461f5-5e73-4f2e-8c1e-4358d4d6f46c#4
EndFittingKey: v3#c5e461f5-5e73-4f2e-8c1e-4358d4d6f46c#4
Name: JIS K 6741/JIS K 6739 - Jointed PVC-U Pipe and Fittings
Schedule: VP
IntermediateSegmentsMax: 2500 mm
TerminationSegmentsMax: 2500 mm
PipeKey: v3#45338dd0-af69-48c0-a2ed-8ade33a08701#5
CouplingKey: v3#eaa8de87-dc67-4eca-ba7e-4267a30f8f7f#2
Elbow90Key: v3#c4513a61-3106-4a78-baf9-a1badd100245#2
Elbow45Key: v3#2769403e-a4fd-4a4c-8e4c-659ea845bd78#2
_ComponentInfo: <CS><C N="Pipe" R="2.400000" IR="2.040000" PL="PL" PN="JIS K 6741 Pipe VP 40"><CO N="1"><FE V="0"/><FD V="1"/><ET V="Jointed"/><NS V="M40"/><MA  V="4.000000"/><MI V="0.800000"/><WP X="0.000000" Y="0.000000" Z="0.000000"/><WA X="-1.000000" Y="0.000000" Z="0.000000"/></CO><CO N="2"><FE  V="0"/><FD V="0"/><ET V="Jointed"/><NS V="M40"/><MA V="4.000000"/><MI V="0.800000"/><WP X="-25.000000" Y="0.000000" Z="0.000000"/><WA X="-1.000000"  Y="0.000000" Z="0.000000"/></CO></C><C N="Coupling" CW="4.700000"><CO N="1"><FE V="1"/><FD V="1"/><ET V="Jointed"/><NS V="M40"/><MA V="2.200000"/><MI  V="0.440000"/><WP X="0.000000" Y="0.000000" Z="0.000000"/><WA X="1.000000" Y="0.000000" Z="0.000000"/></CO><CO N="2"><FE V="1"/><FD V="0"/><ET  V="Jointed"/><NS V="M40"/><MA V="2.200000"/><MI V="0.440000"/><WP X="4.700000" Y="0.000000" Z="0.000000"/><WA X="1.000000" Y="0.000000"  Z="0.000000"/></CO></C><C N="Elbow90" ER="2.700000" S1="4.900000" S2="4.900000" D1="2.200000" D2="2.200000"><CO N="1"><FE V="1"/><FD V="1"/><ET  V="Jointed"/><NS V="M40"/><MA V="2.200000"/><MI V="0.440000"/><WP X="4.900000" Y="0.000000" Z="4.900000"/><WA X="-1.000000" Y="0.000000"  Z="0.000000"/></CO><CO N="2"><FE V="1"/><FD V="0"/><ET V="Jointed"/><NS V="M40"/><MA V="2.200000"/><MI V="0.440000"/><WP X="0.000000" Y="0.000000"  Z="0.000000"/><WA X="0.000000" Y="0.000000" Z="-1.000000"/></CO></C><C N="Elbow45" ER="3.379899" S1="3.600000" S2="3.600000" D1="2.200000"  D2="2.200000"><CO N="1"><FE V="1"/><FD V="1"/><ET V="Jointed"/><NS V="M40"/><MA V="2.200000"/><MI V="0.440000"/><WP X="2.545584" Y="0.000000"  Z="6.145584"/><WA X="-0.707107" Y="0.000000" Z="-0.707107"/></CO><CO N="2"><FE V="1"/><FD V="0"/><ET V="Jointed"/><NS V="M40"/><MA V="2.200000"/><MI  V="0.440000"/><WP X="0.000000" Y="0.000000" Z="0.000000"/><WA X="0.000000" Y="0.000000" Z="-1.000000"/></CO></C></CS>
Name: Hydraulic Hose - Male Straight Thread
_ComponentInfo: <CS><C N="Pipe" R="1.117600" OR="1.117600" IR="0.635000" PL="PL" PartType="" SymKey="" PN="Parker Hydraulic Hose - No Skive 1/2"><CO N="1"><FE V="0"/><FD V="0"/><ET V="Hose - Permanent"/><NS V="1/2"/><MA V="2.540000"/><MI V="0.508000"/><WP X="12.700000" Y="0.000000" Z="0.000000"/><WA X="1.000000" Y="0.000000" Z="0.000000"/></CO><CO N="2"><FE V="0"/><FD V="1"/><ET V="Hose - Permanent"/><NS V="1/2"/><MA V="2.540000"/><MI V="0.508000"/><WP X="0.000000" Y="0.000000" Z="0.000000"/><WA X="1.000000" Y="0.000000" Z="0.000000"/></CO></C><C N="StartFitting" PartType="MISC-HYGENIC" SymKey="ADMF"><CO N="1"><FE V="0"/><FD V="1"/><ET V="Threaded"/><NS V="3/4-16 UNF"/><MA V="1.072520"/><MI V="0.214504"/><WP X="0.000000" Y="0.000000" Z="0.000000"/><WA X="1.000000" Y="0.000000" Z="0.000000"/></CO><CO N="2"><FE V="1"/><FD V="0"/><ET V="Hose - Permanent"/><NS V="1/2"/><MA V="3.200400"/><MI V="3.200400"/><WP X="6.248400" Y="0.000000" Z="0.000000"/><WA X="1.000000" Y="0.000000" Z="0.000000"/></CO></C><C N="EndFitting" PartType="MISC-HYGENIC" SymKey="ADMF"><CO N="1"><FE V="0"/><FD V="1"/><ET V="Threaded"/><NS V="3/4-16 UNF"/><MA V="1.072520"/><MI V="0.214504"/><WP X="0.000000" Y="0.000000" Z="0.000000"/><WA X="1.000000" Y="0.000000" Z="0.000000"/></CO><CO N="2"><FE V="1"/><FD V="0"/><ET V="Hose - Permanent"/><NS V="1/2"/><MA V="3.200400"/><MI V="3.200400"/><WP X="6.248400" Y="0.000000" Z="0.000000"/><WA X="1.000000" Y="0.000000" Z="0.000000"/></CO></C></CS>
StartFittingKey: v3#b50cb43e-68c0-48ac-8e25-7ef224ce0e6c#3
EndFittingKey: v3#b50cb43e-68c0-48ac-8e25-7ef224ce0e6c#3
Name: DIN 8062/DIN 8063 - Jointed PVC-U Pipe and Fittings
Schedule: 6.3
PipeKey: v3#3d294dc7-89c3-4c37-a0ae-28c15a73bfd0#13
CouplingKey: v3#3edf83e2-464b-4b31-84c5-c329ffbf2a4f#5
Elbow90Key: v3#fbd68fd5-590c-4cb5-8c20-9e9bdd396a04#5
Elbow45Key: v3#2f597a97-b15b-49d4-87cb-7bfe69eb62ee#5
_ComponentInfo: <CS><C N="Pipe" R="2.000000" IR="1.700000" PL="PL" PN="DIN 8062 Pipe 40 x 3"><CO N="1"><FE V="0"/><FD V="0"/><ET V="Jointed"/><NS V="M40"/><MA  V="8.000000"/><MI V="1.600000"/><WP X="25.000000" Y="0.000000" Z="0.000000"/><WA X="1.000000" Y="0.000000" Z="0.000000"/></CO><CO N="2"><FE  V="0"/><FD V="1"/><ET V="Jointed"/><NS V="M40"/><MA V="8.000000"/><MI V="1.600000"/><WP X="0.000000" Y="0.000000" Z="0.000000"/><WA X="1.000000"  Y="0.000000" Z="0.000000"/></CO></C><C N="Coupling" CW="5.500000"><CO N="1"><FE V="1"/><FD V="1"/><ET V="Jointed"/><NS V="M40"/><MA V="2.600000"/><MI  V="0.520000"/><WP X="0.000000" Y="0.000000" Z="0.000000"/><WA X="1.000000" Y="0.000000" Z="0.000000"/></CO><CO N="2"><FE V="1"/><FD V="0"/><ET  V="Jointed"/><NS V="M40"/><MA V="2.600000"/><MI V="0.520000"/><WP X="5.500000" Y="0.000000" Z="0.000000"/><WA X="1.000000" Y="0.000000"  Z="0.000000"/></CO></C><C N="Elbow90" ER="8.000000" S1="10.600000" S2="10.600000" D1="2.600000" D2="2.600000"><CO N="1"><FE V="1"/><FD V="0"/><ET  V="Jointed"/><NS V="M40"/><MA V="2.600000"/><MI V="0.520000"/><WP X="10.600000" Y="0.000000" Z="10.600000"/><WA X="1.000000" Y="0.000000"  Z="-0.000000"/></CO><CO N="2"><FE V="1"/><FD V="0"/><ET V="Jointed"/><NS V="M40"/><MA V="2.600000"/><MI V="0.520000"/><WP X="0.000000" Y="0.000000"  Z="-0.000000"/><WA X="-0.000000" Y="0.000000" Z="-1.000000"/></CO></C><C N="Elbow45" ER="2.293503" S1="3.550000" S2="3.550000" D1="2.600000"  D2="2.600000"><CO N="1"><FE V="1"/><FD V="0"/><ET V="Jointed"/><NS V="M40"/><MA V="2.600000"/><MI V="0.520000"/><WP X="2.510229" Y="0.000000"  Z="6.060229"/><WA X="0.707107" Y="0.000000" Z="0.707107"/></CO><CO N="2"><FE V="1"/><FD V="0"/><ET V="Jointed"/><NS V="M40"/><MA V="2.600000"/><MI  V="0.520000"/><WP X="0.000000" Y="0.000000" Z="0.000000"/><WA X="-0.000000" Y="0.000000" Z="-1.000000"/></CO></C></CS>
count: 30
Refkey_Axis1_Context: 2|0|0|0|1|0|0|0|
Refkey_Axis1: 6|0|0|0|44|0|0|0|78|0|65|0|77|0|69|0|83|0|10|0|67|0|111|0|108|0|111|0|114|0|115|0|10|0|49|0|58|0|10|0|10|0|69|0|78|0|68|0|10|0|0|0|
Refkey_Axis2_Context: 2|0|0|0|1|0|0|0|
Refkey_Axis2: 6|0|0|0|88|0|0|0|78|0|65|0|77|0|69|0|83|0|10|0|67|0|111|0|108|0|111|0|114|0|115|0|10|0|49|0|58|0|82|0|111|0|117|0|116|0|101|0|32|0|85|0|73|0|32|0|84|0|111|0|111|0|108|0|32|0|40|0|65|0|120|0|105|0|115|0|32|0|50|0|41|0|10|0|10|0|69|0|78|0|68|0|10|0|0|0|
Refkey_Axis3_Context: 2|0|0|0|1|0|0|0|
Refkey_Axis3: 6|0|0|0|88|0|0|0|78|0|65|0|77|0|69|0|83|0|10|0|67|0|111|0|108|0|111|0|114|0|115|0|10|0|49|0|58|0|82|0|111|0|117|0|116|0|101|0|32|0|85|0|73|0|32|0|84|0|111|0|111|0|108|0|32|0|40|0|65|0|120|0|105|0|115|0|32|0|51|0|41|0|10|0|10|0|69|0|78|0|68|0|10|0|0|0|
Refkey_Ext_Context: 2|0|0|0|1|0|0|0|
Refkey_Ext: 6|0|0|0|92|0|0|0|78|0|65|0|77|0|69|0|83|0|10|0|67|0|111|0|108|0|111|0|114|0|115|0|10|0|49|0|58|0|82|0|111|0|117|0|116|0|101|0|32|0|85|0|73|0|32|0|84|0|111|0|111|0|108|0|32|0|40|0|69|0|120|0|116|0|101|0|110|0|100|0|101|0|114|0|41|0|10|0|10|0|69|0|78|0|68|0|10|0|0|0|
Refkey_Snap_Context: 2|0|0|0|1|0|0|0|
Refkey_Snap: 6|0|0|0|84|0|0|0|78|0|65|0|77|0|69|0|83|0|10|0|67|0|111|0|108|0|111|0|114|0|115|0|10|0|49|0|58|0|82|0|111|0|117|0|116|0|101|0|32|0|85|0|73|0|32|0|84|0|111|0|111|0|108|0|32|0|40|0|83|0|110|0|97|0|112|0|41|0|10|0|10|0|69|0|78|0|68|0|10|0|0|0|